# Autodesk Inventor assembly: full_assembly
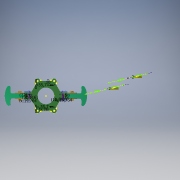
[picture p0: Inventor's stored thumbnail of the model, 180x180]
Saved by Autodesk Inventor 2019 (Build 230136000, 136)
## iProperties
Created: 2021-01-29
Part Number: full_assembly
Material: Genérico
Document SubType Name: Assembly
Designer: Juan M. Casillas
Author: Juan M. Casillas
## Documents named in this file (4)
- K:\3DPrinting\3DModels\shifter\full_assembly.iam
- K:\3DPrinting\3DModels\shifter\plate.ipt
- K:\3DPrinting\3DModels\shifter\lever_group.iam
- K:\3DPrinting\3DModels\shifter\reinforce.ipt
## Components (5 placed, 3 different names)
1. plate:1 — Rigid:1, Rigid:2
2. lever_group:1 [sub-assembly] — Rigid:1
3. lever_group:2 [sub-assembly] — Rigid:2
4. reinforce:1
5. reinforce:2
## Relationships (2: WeldJoint 2)
- Rigid:1 [WeldJoint]: plate:1 ↔ lever_group:1
- Rigid:2 [WeldJoint]: plate:1 ↔ lever_group:2
